# Autodesk Inventor assembly: 00126334_BA-281709-F-7024
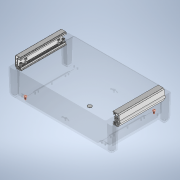
[picture p0: Inventor's stored thumbnail of the model, 180x180]
Saved by Autodesk Inventor 2021 (Build 250183000, 183)
## iProperties
Created: 2019-04-17
Part Number: 00126334_BA-281709-F-7024
Document SubType Name: Assembly
Designer: lgnds
Sending System: Autodesk Inventor 2018
Preprocessor: ST-DEVELOPER v16.13
Title: F:\User\Daten\DWG\Anw\FW\Zwischenspeicher\BA 281709-F.stp
Author: watermann
## Documents named in this file (7)
- C:\Users\Viktor Lindström\Documents\GitHub\WaveRunner-CCU\CCU_Assembly\hw\CAD\Box\00126334_BA-281709-F-7024.iam
- C:\Users\Viktor Lindström\Documents\GitHub\WaveRunner-CCU\CCU_Assembly\hw\CAD\Box\BA 281709 UT.ipt
- C:\Users\Viktor Lindström\Documents\GitHub\WaveRunner-CCU\CCU_Assembly\hw\CAD\Box\BA-17-AP.iam
- C:\Users\Viktor Lindström\Documents\GitHub\WaveRunner-CCU\CCU_Assembly\hw\CAD\Box\BA-17-SP.iam
- C:\Users\Viktor Lindström\Documents\GitHub\WaveRunner-CCU\CCU_Assembly\hw\CAD\Box\SHR Z M4x10,5x4 TX10.ipt
- C:\Users\Viktor Lindström\Documents\GitHub\WaveRunner-CCU\CCU_Assembly\hw\CAD\Box\SHR Z M4x7 DIN 84 Erdungsschraube verkupfert.ipt
- C:\Users\Viktor Lindström\Documents\GitHub\WaveRunner-CCU\CCU_Assembly\hw\CAD\Other\DAE-D11.ipt
## Components (14 placed, 6 different names)
1. BA 281709 UT:1 — Rigid:1
2. BA-17-AP:1 [sub-assembly]
3. BA-17-SP:1 [sub-assembly]
4. SHR Z M4x10,5x4 TX10:1
5. SHR Z M4x10,5x4 TX10:2
6. SHR Z M4x10,5x4 TX10:3
7. SHR Z M4x10,5x4 TX10:4
8. SHR Z M4x10,5x4 TX10:5
9. SHR Z M4x10,5x4 TX10:6
10. SHR Z M4x10,5x4 TX10:7
11. SHR Z M4x10,5x4 TX10:8
12. SHR Z M4x7 DIN 84 Erdungsschraube verkupfert:1
13. SHR Z M4x7 DIN 84 Erdungsschraube verkupfert:2
14. DAE-D11:1 — Rigid:1
## Relationships (1: WeldJoint 1)
- Rigid:1 [WeldJoint]: BA 281709 UT:1 ↔ DAE-D11:1
